# Autodesk Inventor assembly: motor_assembly
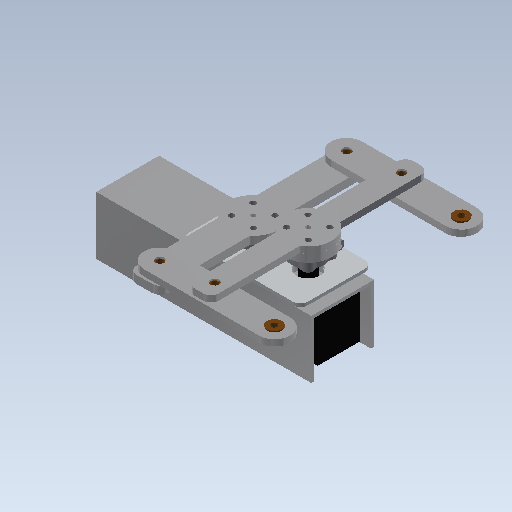
[picture p0: Inventor's stored thumbnail of the model, 512x512]
Saved by Autodesk Inventor 2020 (Build 240168000, 168)
## iProperties
Created: 2017-11-25
Part Number: motor_assembly
Document SubType Name: Assembly
Designer: stedrock
Mass: 181.138 g
Surface Area: 934.212 cm^2
Volume: 181.138 cm^3
Density: 1 g/cm^3
Author: stedrock
## Documents named in this file (12)
- C:\Users\jous\Desktop\boat\motor_assembly.iam
- C:\Users\jous\Desktop\boat\motor.ipt
- C:\Users\jous\Desktop\boat\dhub\dhub.iam
- C:\Users\jous\Desktop\boat\motor_horn.ipt
- C:\Users\jous\Desktop\boat\encoder.ipt
- C:\Users\jous\Desktop\boat\encoder_horn.ipt
- C:\Users\jous\Desktop\boat\motor_base.ipt
- C:\Users\jous\Desktop\boat\H4FM_0405_04.ipt
- C:\Users\jous\Desktop\boat\motor_link.ipt
- C:\Users\jous\Desktop\boat\encoder_spacer.ipt
- C:\Users\jous\Desktop\boat\motor_acrylic_flange1.ipt
- C:\Users\jous\Desktop\boat\motor_acrylic_flange2.ipt
## Components (22 placed, 11 different names)
1. motor:1 — Rotational:2, Rotational:3, Rotational:6, Angle:1
2. dhub:1 [sub-assembly] — Rotational:2, Mate:1
3. motor_horn:1 — Mate:1, Rotational:3, Rotational:8, Rotational:11, Angle:3
4. encoder:1 — Rotational:4, Rotational:5, Rotational:7, Angle:2
5. dhub:2 [sub-assembly] — Rotational:4
6. encoder_horn:1 — Rotational:5, Angle:3, Rotational:19, Rotational:25, Rotational:26
7. motor_base:1 — Rotational:6, Rotational:7, Angle:1, Angle:2, Angle:4, Rotational:27, Angle:6
8. H4FM_0405_04:1 — Rotational:26
9. H4FM_0405_04:2 — Rotational:11, Rotational:24
10. H4FM_0405_04:3 — Rotational:8, Rotational:16
11. H4FM_0405_04:4 — Rotational:19
12. motor_link:1 — Angle:4, Rotational:17, Rotational:18, Rotational:20, Angle:5
13. H4FM_0405_04:7 — Rotational:16, Rotational:17
14. H4FM_0405_04:8 — Rotational:18
15. H4FM_0405_04:9 — Rotational:20
16. motor_link:2 — Angle:5
17. H4FM_0405_04:10 — Rotational:24
18. H4FM_0405_04:11
19. H4FM_0405_04:12
20. encoder_spacer:1 — Rotational:25
21. motor_acrylic_flange1:1 — Rotational:27, Angle:6, Rigid:29
22. motor_acrylic_flange2:1 — Rigid:29
## Relationships (28: RevoluteJoint 20, Angle 6, Mate 1, WeldJoint 1)
- Rotational:2 [RevoluteJoint]: motor:1 ↔ dhub:1
- Mate:1: dhub:1 ↔ motor_horn:1
- Rotational:3 [RevoluteJoint]: motor:1 ↔ motor_horn:1
- Rotational:4 [RevoluteJoint]: encoder:1 ↔ dhub:2
- Rotational:5 [RevoluteJoint] (5 mm): encoder:1 ↔ encoder_horn:1
- Rotational:6 [RevoluteJoint]: motor:1 ↔ motor_base:1
- Rotational:7 [RevoluteJoint]: encoder:1 ↔ motor_base:1
- Angle:1 (180 deg): motor:1 ↔ motor_base:1
- Angle:2 (180 deg): encoder:1 ↔ motor_base:1
- Rotational:8 [RevoluteJoint]: motor_horn:1 ↔ H4FM_0405_04:3
- Rotational:11 [RevoluteJoint]: motor_horn:1 ↔ H4FM_0405_04:2
- Angle:3 (0 deg): motor_horn:1 ↔ encoder_horn:1
- Angle:4 (0 deg): motor_base:1 ↔ motor_link:1
- Rotational:16 [RevoluteJoint]: H4FM_0405_04:3 ↔ H4FM_0405_04:7
- Rotational:17 [RevoluteJoint]: motor_link:1 ↔ H4FM_0405_04:7
- Rotational:18 [RevoluteJoint]: motor_link:1 ↔ H4FM_0405_04:8
- Rotational:19 [RevoluteJoint]: encoder_horn:1 ↔ H4FM_0405_04:4
- Rotational:20 [RevoluteJoint]: motor_link:1 ↔ H4FM_0405_04:9
- [RevoluteJoint]: motor_link:2 ↔ H4FM_0405_04:10
- [RevoluteJoint]: motor_link:2 ↔ H4FM_0405_04:11
- [RevoluteJoint]: motor_link:2 ↔ H4FM_0405_04:12
- Rotational:24 [RevoluteJoint]: H4FM_0405_04:2 ↔ H4FM_0405_04:10
- Angle:5 (180 deg): motor_link:1 ↔ motor_link:2
- Rotational:25 [RevoluteJoint]: encoder_horn:1 ↔ encoder_spacer:1
- Rotational:26 [RevoluteJoint]: encoder_horn:1 ↔ H4FM_0405_04:1
- Rotational:27 [RevoluteJoint]: motor_base:1 ↔ motor_acrylic_flange1:1
- Angle:6 (180 deg): motor_base:1 ↔ motor_acrylic_flange1:1
- Rigid:29 [WeldJoint]: motor_acrylic_flange1:1 ↔ motor_acrylic_flange2:1
## Named parameters: d45_d39 = 0 mm, d46_d40 = 0 deg, d47_d43 = 0 mm, d48_d44 = 0 deg, d49_d37 = 0 mm, d50_d38 = 146.326134 deg
